# Autodesk Inventor assembly: MARCO SP40-01 2100X800
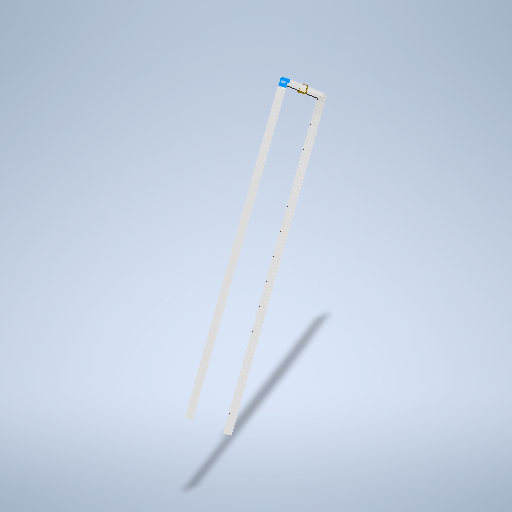
[picture p0: Inventor's stored thumbnail of the model, 512x512]
Saved by Autodesk Inventor 2025 (Build 290162000, 162)
## iProperties
Created: 2026-02-12
Part Number: MARCO SP40-01 2100X800
Document SubType Name: Assembly
Designer: Frank
Author: Frank
## Documents named in this file (9)
- D:\Inventor\Proyectos\MARQUTERIA DE ALUMINIO\MARCOS INTERIOR\MARCO SP40-01 2100X800.iam
- D:\Inventor\Proyectos\MARQUTERIA DE ALUMINIO\MARCOS INTERIOR\SP40-01 MARCO BATIENTE - PAÑO FIJO 800 mm.ipt
- D:\Inventor\Proyectos\MARQUTERIA DE ALUMINIO\MARCOS INTERIOR\JUNTA DE GOMA 800 mm.ipt
- D:\Inventor\Proyectos\MARQUTERIA DE ALUMINIO\MARCOS INTERIOR\BRA-13 ESCUADRA UNIÓN 45 37 mm.ipt
- D:\Inventor\Proyectos\MARQUTERIA DE ALUMINIO\MARCOS INTERIOR\SP40-01 MARCO BATIENTE - PAÑO FIJO 2100 mm.ipt
- D:\Inventor\Proyectos\MARQUTERIA DE ALUMINIO\MARCOS INTERIOR\JUNTA DE GOMA 2100 mm.ipt
- D:\Inventor\Proyectos\MARQUTERIA DE ALUMINIO\MARCOS INTERIOR\SP40-01 MARCO BATIENTE - PAÑO FIJO 2100 mm_MIR.ipt
- D:\Inventor\Proyectos\MARQUTERIA DE ALUMINIO\MARCOS INTERIOR\JUNTA DE GOMA 2100 mm_MIR.ipt
- D:\Inventor\Proyectos\MARQUTERIA DE ALUMINIO\GENERAL\ESCUADRA UNIÓN 45 FINA_MIR1.ipt
## Components (8 placed, 8 different names)
1. SP40-01 MARCO BATIENTE - PAÑO FIJO 800 mm:1 — Coincidencia:1, Coincidencia:2, Coincidencia:3, Coincidencia:6, Coincidencia:7, Coincidencia:8, Coincidencia:12, Coincidencia:13, Coincidencia:19, Coincidencia:20, Coincidencia:21, Coincidencia:22
2. JUNTA DE GOMA 800 mm:1 — Coincidencia:1, Coincidencia:2, Coincidencia:3
3. SP40-01 MARCO BATIENTE - PAÑO FIJO 2100 mm:1 — Coincidencia:6, Coincidencia:7, Coincidencia:8, Coincidencia:9, Coincidencia:10, Coincidencia:11, Coincidencia:14
4. JUNTA DE GOMA 2100 mm:1 — Coincidencia:9, Coincidencia:10, Coincidencia:11
5. BRA-13 ESCUADRA UNIÓN 45 37 mm:1 — Coincidencia:12, Coincidencia:13, Coincidencia:14
6. SP40-01 MARCO BATIENTE - PAÑO FIJO 2100 mm_MIR:1 — Coincidencia:15, Coincidencia:16, Coincidencia:17, Coincidencia:18, Coincidencia:20, Coincidencia:22
7. JUNTA DE GOMA 2100 mm_MIR:1 — Coincidencia:15, Coincidencia:16, Coincidencia:17
8. ESCUADRA UNIÓN 45 FINA_MIR1:1 — Coincidencia:18, Coincidencia:19, Coincidencia:21
## Relationships (20: Mate 20)
- Coincidencia:1 [Mate]: SP40-01 MARCO BATIENTE - PAÑO FIJO 800 mm:1 ↔ JUNTA DE GOMA 800 mm:1
- Coincidencia:2 [Mate]: SP40-01 MARCO BATIENTE - PAÑO FIJO 800 mm:1 ↔ JUNTA DE GOMA 800 mm:1
- Coincidencia:3 [Mate]: SP40-01 MARCO BATIENTE - PAÑO FIJO 800 mm:1 ↔ JUNTA DE GOMA 800 mm:1
- Coincidencia:6 [Mate]: SP40-01 MARCO BATIENTE - PAÑO FIJO 800 mm:1 ↔ SP40-01 MARCO BATIENTE - PAÑO FIJO 2100 mm:1
- Coincidencia:7 [Mate]: SP40-01 MARCO BATIENTE - PAÑO FIJO 800 mm:1 ↔ SP40-01 MARCO BATIENTE - PAÑO FIJO 2100 mm:1
- Coincidencia:8 [Mate]: SP40-01 MARCO BATIENTE - PAÑO FIJO 800 mm:1 ↔ SP40-01 MARCO BATIENTE - PAÑO FIJO 2100 mm:1
- Coincidencia:9 [Mate]: SP40-01 MARCO BATIENTE - PAÑO FIJO 2100 mm:1 ↔ JUNTA DE GOMA 2100 mm:1
- Coincidencia:10 [Mate]: SP40-01 MARCO BATIENTE - PAÑO FIJO 2100 mm:1 ↔ JUNTA DE GOMA 2100 mm:1
- Coincidencia:11 [Mate]: SP40-01 MARCO BATIENTE - PAÑO FIJO 2100 mm:1 ↔ JUNTA DE GOMA 2100 mm:1
- Coincidencia:12 [Mate]: SP40-01 MARCO BATIENTE - PAÑO FIJO 800 mm:1 ↔ BRA-13 ESCUADRA UNIÓN 45 37 mm:1
- Coincidencia:13 [Mate] (1 mm): SP40-01 MARCO BATIENTE - PAÑO FIJO 800 mm:1 ↔ BRA-13 ESCUADRA UNIÓN 45 37 mm:1
- Coincidencia:14 [Mate]: SP40-01 MARCO BATIENTE - PAÑO FIJO 2100 mm:1 ↔ BRA-13 ESCUADRA UNIÓN 45 37 mm:1
- Coincidencia:15 [Mate]: SP40-01 MARCO BATIENTE - PAÑO FIJO 2100 mm_MIR:1 ↔ JUNTA DE GOMA 2100 mm_MIR:1
- Coincidencia:16 [Mate]: SP40-01 MARCO BATIENTE - PAÑO FIJO 2100 mm_MIR:1 ↔ JUNTA DE GOMA 2100 mm_MIR:1
- Coincidencia:17 [Mate]: SP40-01 MARCO BATIENTE - PAÑO FIJO 2100 mm_MIR:1 ↔ JUNTA DE GOMA 2100 mm_MIR:1
- Coincidencia:18 [Mate]: SP40-01 MARCO BATIENTE - PAÑO FIJO 2100 mm_MIR:1 ↔ ESCUADRA UNIÓN 45 FINA_MIR1:1
- Coincidencia:19 [Mate]: SP40-01 MARCO BATIENTE - PAÑO FIJO 800 mm:1 ↔ ESCUADRA UNIÓN 45 FINA_MIR1:1
- Coincidencia:20 [Mate]: SP40-01 MARCO BATIENTE - PAÑO FIJO 800 mm:1 ↔ SP40-01 MARCO BATIENTE - PAÑO FIJO 2100 mm_MIR:1
- Coincidencia:21 [Mate] (1 mm): SP40-01 MARCO BATIENTE - PAÑO FIJO 800 mm:1 ↔ ESCUADRA UNIÓN 45 FINA_MIR1:1
- Coincidencia:22 [Mate]: SP40-01 MARCO BATIENTE - PAÑO FIJO 800 mm:1 ↔ SP40-01 MARCO BATIENTE - PAÑO FIJO 2100 mm_MIR:1
